# Autodesk Inventor assembly: M178-PHTM-2000-01
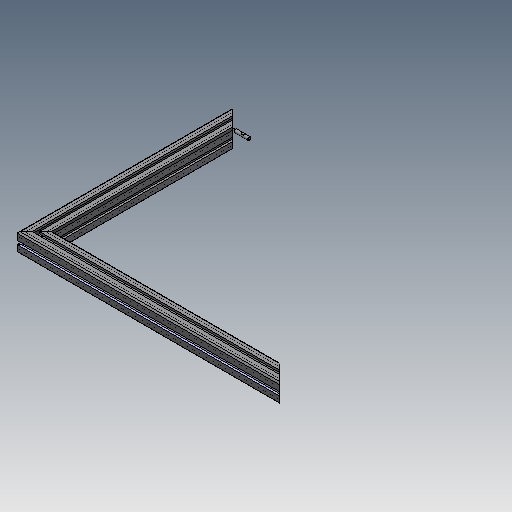
[picture p0: Inventor's stored thumbnail of the model, 512x512]
Saved by Autodesk Inventor 2018.3 (Build 223284000, 284)
## iProperties
Created: 2004-11-19
Part Number: M178-PHTM-2000-01
Document SubType Name: Assembly
Designer: Autodesk, Inc.
Manufacturer: Standard
Standards Organization: Custom
Description: PHANTOM, CABINET BASE ANGLE
Mass: 1392.79 g
Surface Area: 5653.03 cm^2
Volume: 515.589 cm^3
Density: 2.70136 g/cm^3
CAGE: 1LJX3
Dept. ID: Product Design
Description #2: ---
Finish #1: ---
Finish #2: ---
Material ID: ---
Project Number: ---
Author: Autodesk, Inc.
## Documents named in this file (7)
- C:\AVAInvAPI\Workspace\Test Station\Components\M178-2000-Base_Phantom.iam
- C:\AVAInvAPI\Workspace\Test Station\Components\M178-2003.ipt
- C:\AVAInvAPI\Workspace\Test Station\Components\M178-2004.ipt
- C:\AVAInvAPI\Workspace\Test Station\Components\20-128 Mitre Connector.ipt
- C:\AVAInvAPI\Workspace\Test Station\Components\24-506-6F.ipt
- C:\Users\kelleyb.ADS\Desktop\Samples MIGRATED 2009 224 RTM_1\Standard Parts\Test Station Content\Fastners\24-5XX-YY Setscrews.ipt
- C:\Users\kelleyb.ADS\Desktop\Samples MIGRATED 2009 224 RTM_1\Standard Parts\Test Station Content\Extrusions\40 Series Profiles.ipt
## Components (8 placed, 4 different names)
1. 24-506-6F:1
2. 24-506-6F:2
3. 24-506-6F:3
4. 24-506-6F:4
5. M178-2003:1
6. M178-2004:2
7. 20-128 Mitre Connector:1
8. 20-128 Mitre Connector:2
## Relationships (13: Mate 7, Insert 4, Flush 1, Angle 1)
- [Insert]: 24-506-6F:1 ↔ M178-2004:2
- [Insert]: 24-506-6F:2 ↔ M178-2004:2
- [Insert]: 24-506-6F:3 ↔ M178-2003:1
- [Insert]: 24-506-6F:4 ↔ M178-2003:1
- [Flush]: M178-2003:1 ↔ M178-2004:2
- [Mate]: M178-2003:1 ↔ M178-2004:2
- [Mate]: M178-2003:1 ↔ 20-128 Mitre Connector:1
- [Mate]: M178-2003:1 ↔ 20-128 Mitre Connector:1
- [Mate]: M178-2004:2 ↔ 20-128 Mitre Connector:1
- [Angle] (0 deg): M178-2004:2 ↔ 20-128 Mitre Connector:1
- [Mate]: M178-2004:2 ↔ 20-128 Mitre Connector:1
- [Mate]: M178-2004:2 ↔ 20-128 Mitre Connector:2
- [Mate]: M178-2004:2 ↔ 20-128 Mitre Connector:2
